# Autodesk Inventor assembly: DJB_v2_Flex
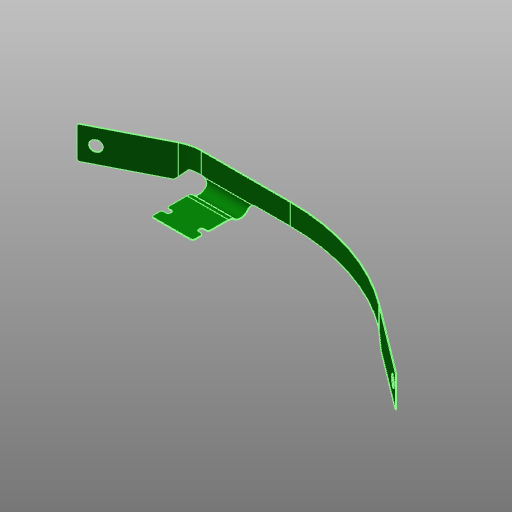
[picture p0: Inventor's stored thumbnail of the model, 512x512]
Saved by Autodesk Inventor 2020.2 (Build 242310000, 310)
## iProperties
Created: 2019-12-30
Part Number: DJB_v2_Flex
Document SubType Name: Assembly
Designer: Mark.Neilson
Mass: 0.0141586 g
Surface Area: 2.90929 cm^2
Volume: 0.0121722 cm^3
Density: 1.16319 g/cm^3
Author: Mark.Neilson
## Documents named in this file (5)
- C:\Users\Mark.Neilson\Desktop\200226\DJB_v2_Flex.iam
- B:\!!Work\Engineering\Inventor\Vendors\Microphones\Sonion\MEMS\O-Series\MEMS_O8XC03.iam
- C:\Users\Mark.Neilson\Desktop\200226\djb_v2_flex_Flex.ipt
- B:\!!Work\Engineering\Inventor\Vendors\Circuits\CerCaps0402.ipt
- B:\!!Work\Engineering\Inventor\WorkInProgress\!!!Review\Harinath Garudadri\191220\CAD files\DJB_Rev2\djb_v2_flex_FlexConnector.ipt
## Components (6 placed, 4 different names)
1. djb_v2_flex_Flex.ipt:1 — Mate:1, Flush:1, Flush:2, Mate:2, Flush:3, Flush:4, Mate:3, Flush:5, Flush:6, Mate:4, Flush:7, Flush:8, Flush:9, Flush:10, Mate:5, Flush:11, Mate:6, Flush:12
2. MEMS_O8XC03.iam:2 [sub-assembly] — Mate:1, Flush:1, Flush:2
3. MEMS_O8XC03.iam:3 [sub-assembly] — Mate:2, Flush:3, Flush:4
4. CerCaps0402.ipt:4 — Mate:3, Flush:5, Flush:6
5. CerCaps0402.ipt:5 — Mate:4, Flush:7, Mate:5
6. djb_v2_flex_FlexConnector.ipt:6 — Flush:11, Mate:6, Flush:12
## Relationships (18: Flush 12, Mate 6)
- Mate:1: djb_v2_flex_Flex.ipt:1 ↔ MEMS_O8XC03.iam:2
- Flush:1: djb_v2_flex_Flex.ipt:1 ↔ MEMS_O8XC03.iam:2
- Flush:2: djb_v2_flex_Flex.ipt:1 ↔ MEMS_O8XC03.iam:2
- Mate:2: djb_v2_flex_Flex.ipt:1 ↔ MEMS_O8XC03.iam:3
- Flush:3: djb_v2_flex_Flex.ipt:1 ↔ MEMS_O8XC03.iam:3
- Flush:4: djb_v2_flex_Flex.ipt:1 ↔ MEMS_O8XC03.iam:3
- Mate:3: djb_v2_flex_Flex.ipt:1 ↔ CerCaps0402.ipt:4
- Flush:5 (1.4859 mm): djb_v2_flex_Flex.ipt:1 ↔ CerCaps0402.ipt:4
- Flush:6 (5.207 mm): djb_v2_flex_Flex.ipt:1 ↔ CerCaps0402.ipt:4
- Mate:4: djb_v2_flex_Flex.ipt:1 ↔ CerCaps0402.ipt:5
- Flush:7 (1.016 mm): djb_v2_flex_Flex.ipt:1 ↔ CerCaps0402.ipt:5
- Flush:8: djb_v2_flex_Flex.ipt:1
- Flush:9: djb_v2_flex_Flex.ipt:1
- Flush:10: djb_v2_flex_Flex.ipt:1
- Mate:5 (-5.1816 mm): djb_v2_flex_Flex.ipt:1 ↔ CerCaps0402.ipt:5
- Flush:11: djb_v2_flex_Flex.ipt:1 ↔ djb_v2_flex_FlexConnector.ipt:6
- Mate:6: djb_v2_flex_Flex.ipt:1 ↔ djb_v2_flex_FlexConnector.ipt:6
- Flush:12: djb_v2_flex_Flex.ipt:1 ↔ djb_v2_flex_FlexConnector.ipt:6
